# Autodesk Inventor assembly: Kegelrad
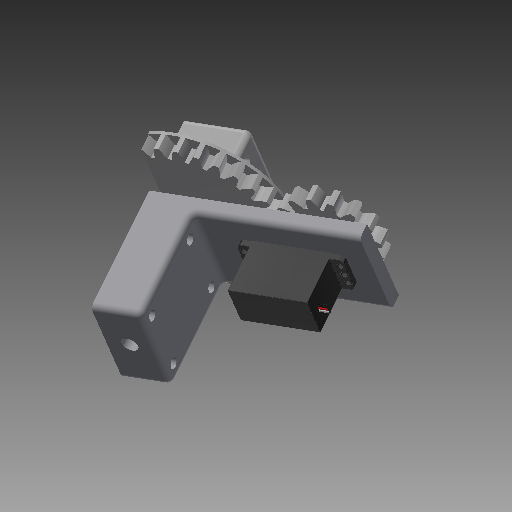
[picture p0: Inventor's stored thumbnail of the model, 512x512]
Saved by Autodesk Inventor 2018 (Build 220112000, 112)
## iProperties
Created: 2018-01-26
Part Number: Kegelrad
Material: Generisch
Document SubType Name: Assembly
Designer: gchri
Author: gchri
## Documents named in this file (4)
- C:\Users\Chris\OneDrive\Development\Mohne\03_Konstruktion\StirnradUNDServo.iam
- C:\Users\Chris\OneDrive\Development\Mohne\03_Konstruktion\StirnradUNDServo\Konstruktions-Assistent\Stirnräder1.iam
- C:\Users\Chris\OneDrive\Development\Mohne\03_Konstruktion\servo_SM-S2309S.ipt
- C:\Users\Chris\OneDrive\Development\Mohne\03_Konstruktion\L-Halterung Servo.ipt
## Components (3 placed, 3 different names)
1. Stirnräder:1 [sub-assembly] — Passend:4, Passend:5
2. servo_SM-S2309S:1 — Passend:1, Passend:2, Passend:3, Passend:4, Passend:5
3. L-Halterung Servo:1 — Passend:1, Passend:2, Passend:3
## Relationships (5: Mate 5)
- Passend:1 [Mate]: servo_SM-S2309S:1 ↔ L-Halterung Servo:1
- Passend:2 [Mate]: servo_SM-S2309S:1 ↔ L-Halterung Servo:1
- Passend:3 [Mate]: servo_SM-S2309S:1 ↔ L-Halterung Servo:1
- Passend:4 [Mate]: Stirnräder:1 ↔ servo_SM-S2309S:1
- Passend:5 [Mate]: Stirnräder:1 ↔ servo_SM-S2309S:1
